# Autodesk Inventor assembly: p1
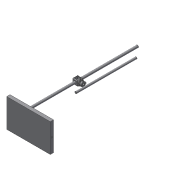
[picture p0: Inventor's stored thumbnail of the model, 180x180]
Saved by Autodesk Inventor 2017 (Build 210142000, 142)
## iProperties
Created: 2021-08-28
Part Number: p1
Document SubType Name: Assembly
Designer: jwoods
Author: jwoods
## Documents named in this file (5)
- C:\work\geothermal-atmospheric-power-generation\experiments\4-Pendulum\mech\p1.iam
- C:\work\geothermal-atmospheric-power-generation\experiments\4-Pendulum\mech\teststand.ipt
- C:\work\geothermal-atmospheric-power-generation\experiments\4-Pendulum\mech\glasstube_1.ipt
- C:\work\geothermal-atmospheric-power-generation\experiments\4-Pendulum\mech\bearing_1.ipt
- C:\work\geothermal-atmospheric-power-generation\experiments\4-Pendulum\mech\bearingtostandsupport.ipt
## Components (4 placed, 4 different names)
1. teststand:1 — Insert:2
2. glasstube_1:1
3. bearingtostandsupport:1 — Insert:2, Insert:3
4. bearing_1:1 — Insert:3
## Relationships (2: Insert 2)
- Insert:2 (-304.8 mm): teststand:1 ↔ bearingtostandsupport:1
- Insert:3: bearingtostandsupport:1 ↔ bearing_1:1
